# Autodesk Inventor assembly: Ratchet Sprocket Gears 1764
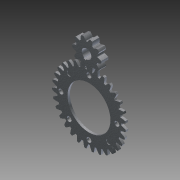
[picture p0: Inventor's stored thumbnail of the model, 180x180]
Saved by Autodesk Inventor 2011 (Build 150239000, 239)
## iProperties
Created: 2010-02-04
Part Number: Ratchet Sprocket Gears 1764
Document SubType Name: Assembly
Designer: jrobinson
Author: jrobinson
## Documents named in this file (3)
- R:\CAD Archives\Manipulators\Ratchet System 1764 Needs Work\Ratchet Sprocket Gears 1764.iam
- R:\CAD Archives\Manipulators\Ratchet System 1764 Needs Work\Spur Gears1.iam
- R:\2009-2010\CAD\Ratchet system\ratchet sprocket gears individual ipts\Design Accelerator\Spur Gear11.ipt
## Components (2 placed, 2 different names)
1. Spur Gears:1 [sub-assembly] — Mate:1, Mate:3, Mate:4
2. Spur Gear1:1 — Mate:1, Mate:3, Mate:4
## Relationships (3: Mate 3)
- Mate:1: Spur Gears:1 ↔ Spur Gear1:1
- Mate:3: Spur Gears:1 ↔ Spur Gear1:1
- Mate:4: Spur Gears:1 ↔ Spur Gear1:1
